# Autodesk Inventor assembly: 217-2000
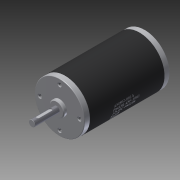
[picture p0: Inventor's stored thumbnail of the model, 180x180]
Saved by Autodesk Inventor 2013 (Build 170138000, 138)
## iProperties
Category: Motors
Company: Autodesk, Inc.
Shininess: 64.0
Length Units: 11272
Angle Units: 11279
Time Units: 11290
Mass Units: 11286
Length Display Precision: 3
Angle Display Precision: 2
Compacted: True
Document SubType Name: Assembly
Created: 2012-12-14
Project: FIRST
Part Number: 217-2000
Description: CIM Motor
Catalog Web Link: http://www.andymark.com/product-p/am-0255.htm
Vendor: AndyMark
Density: 0.0
Volumn: 0.0
Area: 0.0
PropertySet Name: Model Information
Control State: 0
Master: False
Checked Out: False
Title: CIM Motor
Author: Autodesk, Inc.
## Documents named in this file (3)
- E:\Data Folder\FIRST 2013\FIRST KOP\Parts\Motors\MOT_CIM-Motor_217-2000.iam
- E:\Data Folder\FIRST 2013\FIRST KOP\Parts\Motors\FR801-001_CIM Motor Body.ipt
- E:\Data Folder\FIRST 2013\FIRST KOP\Parts\Motors\FR801-001_CIM Motor Machine Screw.ipt
## Components (3 placed, 2 different names)
1. FR801-001_CIM Motor Body:1 — Insert:1, Insert:2
2. FR801-001_CIM Motor Machine Screw:1 — Insert:1
3. FR801-001_CIM Motor Machine Screw:2 — Insert:2
## Relationships (2: Insert 2)
- Insert:1: FR801-001_CIM Motor Body:1 ↔ FR801-001_CIM Motor Machine Screw:1
- Insert:2: FR801-001_CIM Motor Body:1 ↔ FR801-001_CIM Motor Machine Screw:2
